# Autodesk Inventor assembly: PWR_PCB_Assembly
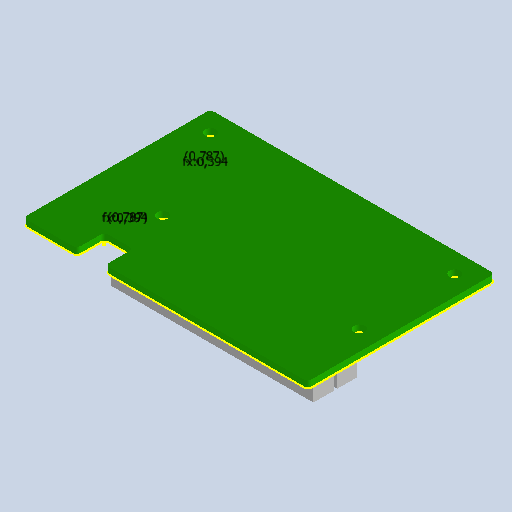
[picture p0: Inventor's stored thumbnail of the model, 512x512]
Saved by Autodesk Inventor 2024.2 (Build 282272000, 272)
## iProperties
Created: 2020-07-14
Part Number: PWR_PCB_Assembly
Document SubType Name: Assembly
Designer: lgnds
Author: lgnds
## Documents named in this file (3)
- C:\Users\lgnds\Documents\GitHub\REACH-Hardware\CAD\InventorProject\PCB_Assemblies\PWR_PCB_Assembly.iam
- C:\Users\lgnds\Documents\GitHub\REACH-Hardware\CAD\InventorProject\PCB_Assemblies\PCB\PWR_PCB.ipt
- C:\Users\lgnds\Documents\GitHub\REACH-Hardware\CAD\InventorProject\PCB_Assemblies\Connector\HLE-120-02-F-DV-BE-A\HLE-120-02-F-DV-BE-A.iam
## Components (3 placed, 3 different names)
1. PWR_PCB:1 — Flush:1, Flush:2, Mate:1, Mate:2
2. HLE-120-02-F-DV-BE-A_NANO:1 [sub-assembly] — Flush:1, Flush:2, Mate:1, Flush:3, Flush:4
3. HLE-120-02-F-DV-BE-A_NX:2 [sub-assembly] — Mate:2, Flush:3, Flush:4
## Relationships (6: Flush 4, Mate 2)
- Flush:1 (1.46 mm): PWR_PCB:1 ↔ HLE-120-02-F-DV-BE-A_NANO:1
- Flush:2: PWR_PCB:1 ↔ HLE-120-02-F-DV-BE-A_NANO:1
- Mate:1: PWR_PCB:1 ↔ HLE-120-02-F-DV-BE-A_NANO:1
- Mate:2: PWR_PCB:1 ↔ HLE-120-02-F-DV-BE-A_NX:2
- Flush:3: HLE-120-02-F-DV-BE-A_NANO:1 ↔ HLE-120-02-F-DV-BE-A_NX:2
- Flush:4 (6 mm): HLE-120-02-F-DV-BE-A_NANO:1 ↔ HLE-120-02-F-DV-BE-A_NX:2
